# Autodesk Inventor assembly: Цепной привод
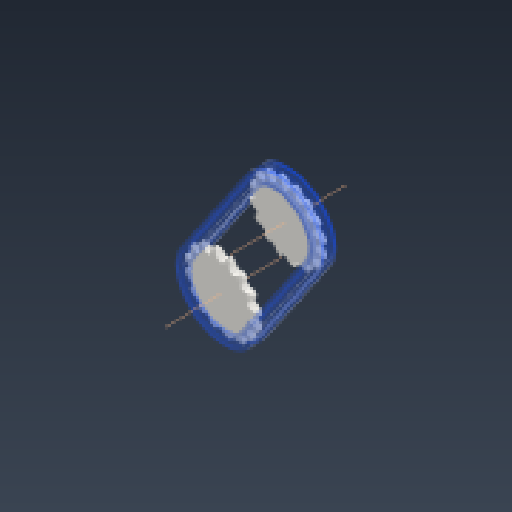
[picture p0: Inventor's stored thumbnail of the model, 512x512]
Saved by Autodesk Inventor 2025 (Build 290162000, 162)
## iProperties
ClientObjectVersion: 1
Created: 2025-03-14
Part Number: Цепной привод
Document SubType Name: Assembly
Designer: GameHD
Author: GameHD
## Documents named in this file (4)
- C:\Users\GameHD\Desktop\phantom 16950\втулка+подшипники нужная сборка\Мастер проектирования\Цепной привод2.iam
- C:\Users\GameHD\Desktop\phantom 16950\втулка+подшипники нужная сборка\Мастер проектирования\Цепь роликовая2.ipt
- C:\Users\GameHD\Desktop\phantom 16950\втулка+подшипники нужная сборка\Мастер проектирования\Звездочка роликовой цепи12.ipt
- C:\Users\GameHD\Desktop\phantom 16950\втулка+подшипники нужная сборка\Мастер проектирования\Звездочка роликовой цепи22.ipt
## Components (3 placed, 3 different names)
1. Цепь роликовая:1 — Заподлицо:1, Совмещение:1, Совмещение:2, Заподлицо:2, Совмещение:3, Совмещение:4
2. Звездочка роликовой цепи1:1 — Заподлицо:1, Совмещение:1, Совмещение:2, ЗубчПер:1
3. Звездочка роликовой цепи2:1 — Заподлицо:2, Совмещение:3, ЗубчПер:1, Совмещение:4
## Relationships (7: Mate 4, Flush 2, RelateRotation 1)
- Заподлицо:1 [Flush]: Цепь роликовая:1 ↔ Звездочка роликовой цепи1:1
- Совмещение:1 [Mate]: Цепь роликовая:1 ↔ Звездочка роликовой цепи1:1
- Совмещение:2 [Mate]: Цепь роликовая:1 ↔ Звездочка роликовой цепи1:1
- Заподлицо:2 [Flush]: Цепь роликовая:1 ↔ Звездочка роликовой цепи2:1
- Совмещение:3 [Mate]: Цепь роликовая:1 ↔ Звездочка роликовой цепи2:1
- ЗубчПер:1 [RelateRotation] (0.6154 ul): Звездочка роликовой цепи1:1 ↔ Звездочка роликовой цепи2:1
- Совмещение:4 [Mate]: Цепь роликовая:1 ↔ Звездочка роликовой цепи2:1
